# Autodesk Inventor assembly: extension arm assembly
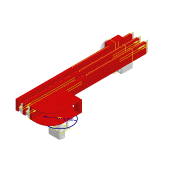
[picture p0: Inventor's stored thumbnail of the model, 180x180]
Saved by Autodesk Inventor 2020 (Build 240168000, 168)
## iProperties
Created: 2020-01-01
Part Number: extension arm assembly
Document SubType Name: Assembly
Designer: ball
Author: ball
## Documents named in this file (6)
- C:\FTC\FTC8863CAD\2019 Robot\Delivery\extension arm\extension arm assembly.iam
- C:\FTC\FTC8863CAD\2019 Robot\Delivery\extension arm\extension arm top.iam
- C:\FTC\FTC8863CAD\2019 Robot\Delivery\extension arm\extension arm middle.iam
- C:\FTC\FTC8863CAD\2019 Robot\Delivery\extension arm\extension arm bottom.iam
- C:\FTC\FTC8863CAD\2019 Robot\Delivery\extension arm\Servo mount + servo.iam
- C:\FTC\FTC8863CAD\2019 Robot\Collection\Collector rotator assembly for extension arm.iam
## Components (5 placed, 5 different names)
1. extension arm top:1 [sub-assembly] — Mate:1, Mate:3, Mate:4, Mate:5, Mate:9, Mate:10, Mate:11, Mate:12
2. extension arm middle:1 [sub-assembly] — Mate:1, Mate:2, Mate:3, Mate:4, Mate:5, Mate:6, Mate:7, Mate:8
3. extension arm bottom:1 [sub-assembly] — Mate:2, Mate:6, Mate:7, Mate:8, Mate:13, Mate:14, Mate:15
4. Servo mount + servo:1 [sub-assembly] — Mate:9, Mate:10, Mate:11, Mate:12
5. Collector rotator assembly for extension arm:1 [sub-assembly] — Mate:13, Mate:14, Mate:15
## Relationships (15: Mate 15)
- Mate:1: extension arm top:1 ↔ extension arm middle:1
- Mate:2: extension arm middle:1 ↔ extension arm bottom:1
- Mate:3: extension arm top:1 ↔ extension arm middle:1
- Mate:4: extension arm top:1 ↔ extension arm middle:1
- Mate:5: extension arm top:1 ↔ extension arm middle:1
- Mate:6: extension arm middle:1 ↔ extension arm bottom:1
- Mate:7: extension arm middle:1 ↔ extension arm bottom:1
- Mate:8: extension arm middle:1 ↔ extension arm bottom:1
- Mate:9: extension arm top:1 ↔ Servo mount + servo:1
- Mate:10: extension arm top:1 ↔ Servo mount + servo:1
- Mate:11: extension arm top:1 ↔ Servo mount + servo:1
- Mate:12: extension arm top:1 ↔ Servo mount + servo:1
- Mate:13: extension arm bottom:1 ↔ Collector rotator assembly for extension arm:1
- Mate:14: extension arm bottom:1 ↔ Collector rotator assembly for extension arm:1
- Mate:15 (0.254 mm): extension arm bottom:1 ↔ Collector rotator assembly for extension arm:1
